# Autodesk Inventor assembly: fixture assembly
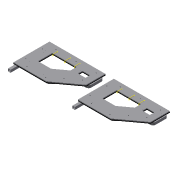
[picture p0: Inventor's stored thumbnail of the model, 180x180]
Saved by Autodesk Inventor 2022 (Build 260148000, 148)
## iProperties
Created: 2006-05-17
Part Number: fixture assembly
Document SubType Name: Assembly
Designer: dchu
Author: dchu
## Documents named in this file (3)
- C:\Autodesk Inventor 2022 Advanced Assembly Modeling Practice Files\iMates\fixture assembly.iam
- C:\Autodesk Inventor 2022 Advanced Assembly Modeling Practice Files\iMates\frame.ipt
- C:\Autodesk Inventor 2022 Advanced Assembly Modeling Practice Files\iMates\plate.ipt
## Components (4 placed, 2 different names)
1. plate:1 — Insert:1, Insert:2
2. frame:1 — Insert:1, Insert:2, Mate:1, Flush:1, Flush:2
3. plate:2 — Insert:3, Insert:4
4. frame:2 — Mate:1, Flush:1, Flush:2, Insert:3, Insert:4
## Relationships (7: Insert 4, Flush 2, Mate 1)
- Insert:1: plate:1 ↔ frame:1
- Insert:2: plate:1 ↔ frame:1
- Mate:1 (1233.282 mm): frame:1 ↔ frame:2
- Flush:1: frame:1 ↔ frame:2
- Flush:2: frame:1 ↔ frame:2
- Insert:3: plate:2 ↔ frame:2
- Insert:4: plate:2 ↔ frame:2
